# Autodesk Inventor assembly: workbench
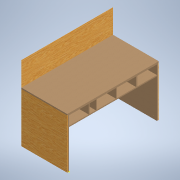
[picture p0: Inventor's stored thumbnail of the model, 180x180]
Saved by Autodesk Inventor 2022 (Build 260153000, 153)
## iProperties
Created: 2022-02-21
Part Number: workbench
Document SubType Name: Assembly
Designer: MarkP
Author: MarkP
## Documents named in this file (16)
- C:\Users\MarkP\Documents\Mark\final\workbench.iam
- C:\Users\MarkP\Documents\Mark\final\desk.ipt
- C:\Users\MarkP\Documents\Mark\final\wallL1.ipt
- C:\Users\MarkP\Documents\Mark\final\wallL2.ipt
- C:\Users\MarkP\Documents\Mark\final\wallL1_MIR.ipt
- C:\Users\MarkP\Documents\Mark\final\wallL2_MIR.ipt
- C:\Users\MarkP\Documents\Mark\final\basedraws.ipt
- C:\Users\MarkP\Documents\Mark\final\reardraws.ipt
- C:\Users\MarkP\Documents\Mark\final\backboard.ipt
- C:\Users\MarkP\Documents\Mark\final\cupboard break.ipt
- C:\Users\MarkP\Documents\Mark\final\workbench\AIP\FEA\dvwk6magw.fins
- C:\Users\MarkP\Documents\Mark\final\workbench\AIP\FEA\dvwk6magw.fsat
- C:\Users\MarkP\Documents\Mark\final\workbench\AIP\FEA\dvwk6magw.ftes
- C:\Users\MarkP\Documents\Mark\final\workbench\AIP\FEA\dvwk6magw.fwiz
- C:\Users\MarkP\Documents\Mark\final\workbench\AIP\FEA\dvwk6maio.fmsh
- C:\Users\MarkP\Documents\Mark\final\workbench\AIP\FEA\dvwk6maip.fres
## Components (12 placed, 9 different names)
1. desk:1 — Mate:2, Flush:3, Mate:3, Flush:6, Mate:7, Mate:9, Flush:9
2. wallL1:1 — Flush:1, Mate:1, Flush:2, Flush:3, Flush:7, Mate:8, Mate:12, Mate:20, Mate:21, Mate:22, Mate:26
3. wallL2:1 — Flush:1, Mate:1, Flush:2, Mate:2, Mate:3, Mate:6, Flush:8
4. wallL1_MIR:1 — Flush:4, Mate:4, Flush:5, Mate:19, Mate:23
5. wallL2_MIR:1 — Flush:4, Mate:4, Flush:5, Mate:5
6. basedraws:1 — Flush:6, Mate:5, Flush:7, Mate:10, Mate:14, Mate:15, Mate:24
7. reardraws:1 — Mate:6, Mate:7, Mate:8, Mate:11, Mate:16, Mate:18, Mate:25
8. backboard:1 — Mate:9, Flush:8, Flush:9
9. cupboard break:1 — Mate:10, Mate:11, Mate:12, Mate:21
10. cupboard break:2 — Mate:15, Mate:16, Mate:20, Mate:22
11. cupboard break:3 — Mate:14, Mate:18, Mate:19, Mate:23
12. cupboard break:4 — Mate:24, Mate:25, Mate:26
## Relationships (33: Mate 24, Flush 9)
- Flush:1: wallL1:1 ↔ wallL2:1
- Mate:1: wallL1:1 ↔ wallL2:1
- Flush:2: wallL1:1 ↔ wallL2:1
- Mate:2: desk:1 ↔ wallL2:1
- Flush:3: desk:1 ↔ wallL1:1
- Mate:3: desk:1 ↔ wallL2:1
- Flush:4: wallL1_MIR:1 ↔ wallL2_MIR:1
- Mate:4: wallL1_MIR:1 ↔ wallL2_MIR:1
- Flush:5: wallL1_MIR:1 ↔ wallL2_MIR:1
- Flush:6: desk:1 ↔ basedraws:1
- Mate:5: wallL2_MIR:1 ↔ basedraws:1
- Flush:7: wallL1:1 ↔ basedraws:1
- Mate:6: wallL2:1 ↔ reardraws:1
- Mate:7: desk:1 ↔ reardraws:1
- Mate:8: wallL1:1 ↔ reardraws:1
- Mate:9: desk:1 ↔ backboard:1
- Flush:8: wallL2:1 ↔ backboard:1
- Flush:9: desk:1 ↔ backboard:1
- Mate:10: basedraws:1 ↔ cupboard break:1
- Mate:11: reardraws:1 ↔ cupboard break:1
- Mate:12 (322 mm): wallL1:1 ↔ cupboard break:1
- Mate:14: basedraws:1 ↔ cupboard break:3
- Mate:15: basedraws:1 ↔ cupboard break:2
- Mate:16: reardraws:1 ↔ cupboard break:2
- Mate:18: reardraws:1 ↔ cupboard break:3
- Mate:19 (322 mm): wallL1_MIR:1 ↔ cupboard break:3
- Mate:20 (440 mm): wallL1:1 ↔ cupboard break:2
- Mate:21 (317 mm): wallL1:1 ↔ cupboard break:1
- Mate:22 (435 mm): wallL1:1 ↔ cupboard break:2
- Mate:23 (317 mm): wallL1_MIR:1 ↔ cupboard break:3
- Mate:24: basedraws:1 ↔ cupboard break:4
- Mate:25: reardraws:1 ↔ cupboard break:4
- Mate:26 (770 mm): wallL1:1 ↔ cupboard break:4
## Named parameters: sa_0 = 50000
note: some values were not read from the file. Shown as the stored number, unit unknown: "sa_0".
